# Autodesk Inventor assembly: Elektronik_Gesamtbaugruppe
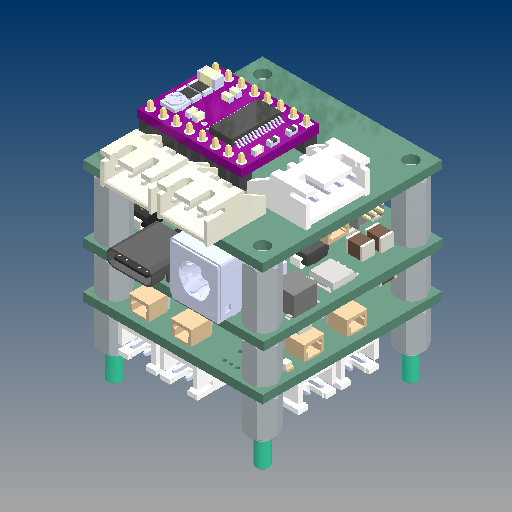
[picture p0: Inventor's stored thumbnail of the model, 512x512]
Saved by Autodesk Inventor 2025 (Build 290162010, 162A)
## iProperties
Created: 2025-02-26
Part Number: Elektronik_Gesamtbaugruppe
Document SubType Name: Assembly
Designer: jan
Author: jan
## Documents named in this file (4)
- C:\Users\jan\Documents\github\fiberprinter-electronics\2nd-mainboard-pcb\export_versions\Elektronik_Gesamtbaugruppe.iam
- C:\Users\jan\Documents\github\fiberprinter-electronics\2nd-mainboard-pcb\export_versions\Modul_Leistung_V2\Modul_Leistung_V2.iam
- C:\Users\jan\Documents\github\fiberprinter-electronics\2nd-mainboard-pcb\export_versions\Modul_Motoren_V2\Modul_Motoren_V2.iam
- C:\Users\jan\Documents\github\fiberprinter-electronics\2nd-mainboard-pcb\export_versions\Modul_Fans\Modul_Fans.iam
## Components (3 placed, 3 different names)
1. Modul_Leistung_V2:1 [sub-assembly] — Passend:1, Passend:2, Passend:3, Passend:4, Passend:5, Passend:6
2. Modul_Motoren_V2:1 [sub-assembly] — Passend:1, Passend:2, Passend:3
3. Modul_Fans:1 [sub-assembly] — Passend:4, Passend:5, Passend:6
## Relationships (6: Mate 6)
- Passend:1 [Mate]: Modul_Leistung_V2:1 ↔ Modul_Motoren_V2:1
- Passend:2 [Mate]: Modul_Leistung_V2:1 ↔ Modul_Motoren_V2:1
- Passend:3 [Mate]: Modul_Leistung_V2:1 ↔ Modul_Motoren_V2:1
- Passend:4 [Mate]: Modul_Leistung_V2:1 ↔ Modul_Fans:1
- Passend:5 [Mate]: Modul_Leistung_V2:1 ↔ Modul_Fans:1
- Passend:6 [Mate]: Modul_Leistung_V2:1 ↔ Modul_Fans:1
